# Autodesk Inventor assembly: Assembly1
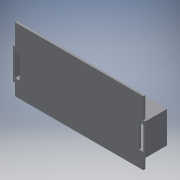
[picture p0: Inventor's stored thumbnail of the model, 180x180]
Saved by Autodesk Inventor 2019 (Build 230136000, 136)
## iProperties
Created: 2019-12-10
Part Number: Assembly1
Document SubType Name: Assembly
Designer: ABHISHEK
Author: ABHISHEK
## Documents named in this file (3)
- D:\team 15\Assembly1.iam
- D:\team 15\Part1.ipt
- D:\team 15\Part2.ipt
## Components (3 placed, 2 different names)
1. Part1:1 — Mate:1, Flush:1, Flush:2, Mate:2, Flush:3, Flush:4
2. Part2:2 — Mate:1, Flush:1, Flush:2
3. Part2:3 — Mate:2, Flush:3, Flush:4
## Relationships (6: Flush 4, Mate 2)
- Mate:1: Part1:1 ↔ Part2:2
- Flush:1: Part1:1 ↔ Part2:2
- Flush:2: Part1:1 ↔ Part2:2
- Mate:2: Part1:1 ↔ Part2:3
- Flush:3: Part1:1 ↔ Part2:3
- Flush:4: Part1:1 ↔ Part2:3
